# Autodesk Inventor assembly: Wash Chamber Conduit Assembly
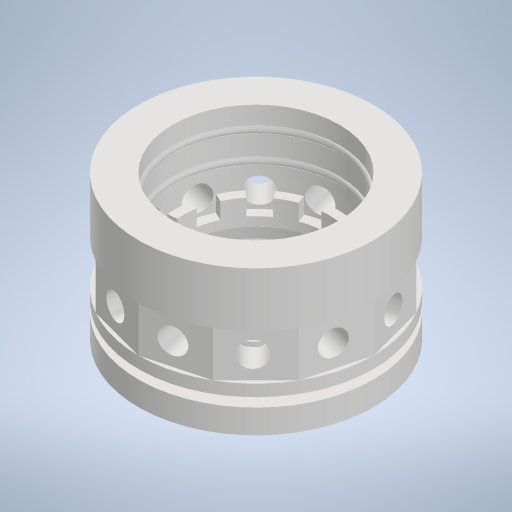
[picture p0: Inventor's stored thumbnail of the model, 512x512]
Saved by Autodesk Inventor 2024 (Build 280153000, 153)
## iProperties
Created: 2024-04-17
Part Number: Wash Chamber Conduit Assembly
Document SubType Name: Assembly
Designer: Tommy Rohmann
Author: Tommy Rohmann
## Documents named in this file (5)
- C:\Users\Tommy Rohmann\Documents\Repositories\Microgravity-Press-Washing-Machine\Sub-System Design and Documentation\3 Wash Chamber Assembly\Wash Chamber Conduit\Wash Chamber Conduit Assembly.iam
- C:\Users\Tommy Rohmann\Documents\Repositories\Microgravity-Press-Washing-Machine\Sub-System Design and Documentation\3 Wash Chamber Assembly\Wash Chamber Conduit\1 Wash Chamber Conduit.ipt
- C:\Users\Tommy Rohmann\Documents\Repositories\Microgravity-Press-Washing-Machine\Sub-System Design and Documentation\3 Wash Chamber Assembly\Wash Chamber Conduit\2 Wash Chamber Conduit External Seal Rings.ipt
- C:\Users\Tommy Rohmann\Documents\Repositories\Microgravity-Press-Washing-Machine\Sub-System Design and Documentation\3 Wash Chamber Assembly\Wash Chamber Conduit\3 Wach Chamber Access Hatch O-Ring.ipt
- C:\Users\Tommy Rohmann\Documents\Repositories\Microgravity-Press-Washing-Machine\Sub-System Design and Documentation\3 Wash Chamber Assembly\Wash Chamber Conduit\4 Castle Spacer.ipt
## Components (6 placed, 4 different names)
1. 1 Wash Chamber Conduit:1 — Mate:1, Tangent:1, Tangent:2, Mate:2, Tangent:3, Mate:3, Tangent:4, Mate:4, Mate:5, Mate:6
2. 2 Wash Chamber Conduit External Seal Rings:1 — Tangent:2, Mate:2
3. 2 Wash Chamber Conduit External Seal Rings:2 — Mate:1, Tangent:1
4. 2 Wash Chamber Conduit External Seal Rings:3 — Tangent:3, Mate:3
5. 3 Wach Chamber Access Hatch O-Ring:1 — Tangent:4, Mate:4
6. 4 Castle Spacer:1 — Mate:5, Mate:6
## Relationships (10: Mate 6, Tangent 4)
- Mate:1: 1 Wash Chamber Conduit:1 ↔ 2 Wash Chamber Conduit External Seal Rings:2
- Tangent:1: 1 Wash Chamber Conduit:1 ↔ 2 Wash Chamber Conduit External Seal Rings:2
- Tangent:2: 1 Wash Chamber Conduit:1 ↔ 2 Wash Chamber Conduit External Seal Rings:1
- Mate:2: 1 Wash Chamber Conduit:1 ↔ 2 Wash Chamber Conduit External Seal Rings:1
- Tangent:3: 1 Wash Chamber Conduit:1 ↔ 2 Wash Chamber Conduit External Seal Rings:3
- Mate:3: 1 Wash Chamber Conduit:1 ↔ 2 Wash Chamber Conduit External Seal Rings:3
- Tangent:4: 1 Wash Chamber Conduit:1 ↔ 3 Wach Chamber Access Hatch O-Ring:1
- Mate:4: 1 Wash Chamber Conduit:1 ↔ 3 Wach Chamber Access Hatch O-Ring:1
- Mate:5: 1 Wash Chamber Conduit:1 ↔ 4 Castle Spacer:1
- Mate:6: 1 Wash Chamber Conduit:1 ↔ 4 Castle Spacer:1
